# Autodesk Inventor assembly: armAssembaly
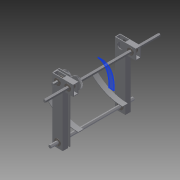
[picture p0: Inventor's stored thumbnail of the model, 180x180]
Saved by Autodesk Inventor 2016 (Build 200138000, 138)
## iProperties
Created: 2016-01-27
Part Number: armAssembaly
Document SubType Name: Assembly
Designer: 278648
Author: 278648
## Documents named in this file (10)
- C:\Users\zachary\Downloads\1510-stronghold-CAD-master\1510-stronghold-CAD-master\pickeruperthingy\armAssembaly.iam
- C:\Users\zachary\Downloads\1510-stronghold-CAD-master\1510-stronghold-CAD-master\pickeruperthingy\arm.ipt
- C:\Users\zachary\Downloads\1510-stronghold-CAD-master\1510-stronghold-CAD-master\pickeruperthingy\217-3875-STEP-20140818.ipt
- C:\Users\zachary\Downloads\1510-stronghold-CAD-master\1510-stronghold-CAD-master\pickeruperthingy\rod.ipt
- C:\Users\zachary\Downloads\1510-stronghold-CAD-master\1510-stronghold-CAD-master\pickeruperthingy\rod2.ipt
- C:\Users\zachary\Downloads\1510-stronghold-CAD-master\1510-stronghold-CAD-master\pickeruperthingy\217-2708.20121204.ipt
- C:\Users\zachary\Downloads\1510-stronghold-CAD-master\1510-stronghold-CAD-master\pickeruperthingy\217-3488-STEP.ipt
- C:\Users\zachary\Downloads\1510-stronghold-CAD-master\1510-stronghold-CAD-master\pickeruperthingy\rod3.ipt
- C:\Users\zachary\Downloads\1510-stronghold-CAD-master\1510-stronghold-CAD-master\pickeruperthingy\Part13.ipt
- C:\Users\zachary\Downloads\1510-stronghold-CAD-master\1510-stronghold-CAD-master\pickeruperthingy\chainguard.ipt
## Components (22 placed, 9 different names)
1. arm:1 — Flush:1, Mate:1, Flush:2, Mate:2, Mate:3, Mate:6, Mate:9, Mate:16, Mate:17, Mate:18, Mate:19, Mate:22, Mate:23, Mate:24, Mate:25, Flush:6, Mate:43, Mate:44, Mate:60, Flush:9, Flush:10, Mate:62
2. arm:2 — Flush:1, Mate:1, Flush:2, Mate:4, Mate:5, Mate:7, Mate:8, Mate:12, Mate:13, Mate:14, Mate:15, Flush:3, Flush:11
3. 217-3875-STEP-20140818:1 — Mate:2, Mate:3, Mate:10, Mate:11
4. 217-3875-STEP-20140818:2 — Mate:4, Mate:5
5. 217-3875-STEP-20140818:3 — Mate:7, Mate:8, Mate:52
6. 217-3875-STEP-20140818:4 — Mate:6, Mate:9, Mate:51
7. rod:1 — Mate:10, Mate:11, Flush:3, Mate:34, Mate:35
8. 217-3875-STEP-20140818:5 — Mate:12, Mate:13
9. 217-3875-STEP-20140818:6 — Mate:14, Mate:15
10. 217-3875-STEP-20140818:7 — Mate:18, Mate:19
11. 217-3875-STEP-20140818:8 — Mate:16, Mate:17, Mate:41, Mate:42
12. 217-3875-STEP-20140818:9 — Mate:22, Mate:23
13. 217-3875-STEP-20140818:12 — Mate:24, Mate:25, Mate:30, Mate:31
14. rod2:2 — Mate:30, Mate:31, Mate:32, Mate:33, Mate:56, Mate:57, Flush:12
15. 217-2708.20121204:1 — Mate:32, Mate:33, Mate:44, Flush:12
16. 217-2708.20121204:2 — Mate:34, Mate:35, Mate:43
17. 217-3488-STEP:1 — Flush:7, Mate:56, Mate:57, Mate:62
18. rod3:1 — Mate:41, Mate:42, Flush:6, Mate:58, Mate:59
19. 217-3488-STEP:2 — Flush:7, Mate:58, Mate:59
20. Part13:1 — Mate:51, Mate:53, Flush:8, Flush:11
21. Part13:2 — Mate:52, Mate:53, Flush:8, Mate:61
22. chainguard:1 — Mate:60, Flush:9, Flush:10, Mate:61
## Relationships (53: Mate 43, Flush 10)
- Flush:1: arm:1 ↔ arm:2
- Mate:1 (279.4 mm): arm:1 ↔ arm:2
- Flush:2: arm:1 ↔ arm:2
- Mate:2: arm:1 ↔ 217-3875-STEP-20140818:1
- Mate:3: arm:1 ↔ 217-3875-STEP-20140818:1
- Mate:4: arm:2 ↔ 217-3875-STEP-20140818:2
- Mate:5: arm:2 ↔ 217-3875-STEP-20140818:2
- Mate:6: arm:1 ↔ 217-3875-STEP-20140818:4
- Mate:7: arm:2 ↔ 217-3875-STEP-20140818:3
- Mate:8: arm:2 ↔ 217-3875-STEP-20140818:3
- Mate:9: arm:1 ↔ 217-3875-STEP-20140818:4
- Mate:10: 217-3875-STEP-20140818:1 ↔ rod:1
- Mate:11: 217-3875-STEP-20140818:1 ↔ rod:1
- Mate:12: arm:2 ↔ 217-3875-STEP-20140818:5
- Mate:13: arm:2 ↔ 217-3875-STEP-20140818:5
- Mate:14: arm:2 ↔ 217-3875-STEP-20140818:6
- Mate:15: arm:2 ↔ 217-3875-STEP-20140818:6
- Mate:16: arm:1 ↔ 217-3875-STEP-20140818:8
- Mate:17: arm:1 ↔ 217-3875-STEP-20140818:8
- Mate:18: arm:1 ↔ 217-3875-STEP-20140818:7
- Mate:19: arm:1 ↔ 217-3875-STEP-20140818:7
- Mate:22: arm:1 ↔ 217-3875-STEP-20140818:9
- Mate:23: arm:1 ↔ 217-3875-STEP-20140818:9
- Mate:24: arm:1 ↔ 217-3875-STEP-20140818:12
- Mate:25: arm:1 ↔ 217-3875-STEP-20140818:12
- Flush:3 (-114.3 mm): arm:2 ↔ rod:1
- Mate:30: 217-3875-STEP-20140818:12 ↔ rod2:2
- Mate:31: 217-3875-STEP-20140818:12 ↔ rod2:2
- Mate:32: rod2:2 ↔ 217-2708.20121204:1
- Mate:33: rod2:2 ↔ 217-2708.20121204:1
- Mate:34: rod:1 ↔ 217-2708.20121204:2
- Mate:35: rod:1 ↔ 217-2708.20121204:2
- Mate:41: 217-3875-STEP-20140818:8 ↔ rod3:1
- Mate:42: 217-3875-STEP-20140818:8 ↔ rod3:1
- Flush:6 (-38.1 mm): arm:1 ↔ rod3:1
- Mate:43 (12.7 mm): arm:1 ↔ 217-2708.20121204:2
- Mate:44 (12.7 mm): arm:1 ↔ 217-2708.20121204:1
- Flush:7: 217-3488-STEP:1 ↔ 217-3488-STEP:2
- Mate:51: 217-3875-STEP-20140818:4 ↔ Part13:1
- Mate:52: 217-3875-STEP-20140818:3 ↔ Part13:2
- Mate:53 (190.5 mm): Part13:1 ↔ Part13:2
- Flush:8: Part13:1 ↔ Part13:2
- Mate:56: rod2:2 ↔ 217-3488-STEP:1
- Mate:57: rod2:2 ↔ 217-3488-STEP:1
- Mate:58: rod3:1 ↔ 217-3488-STEP:2
- Mate:59: rod3:1 ↔ 217-3488-STEP:2
- Mate:60 (8.255 mm): arm:1 ↔ chainguard:1
- Flush:9: arm:1 ↔ chainguard:1
- Flush:10: arm:1 ↔ chainguard:1
- Mate:61 (13.335 mm): Part13:2 ↔ chainguard:1
- Mate:62 (3.175 mm): arm:1 ↔ 217-3488-STEP:1
- Flush:11 (25.4 mm): arm:2 ↔ Part13:1
- Flush:12 (-3.175 mm): rod2:2 ↔ 217-2708.20121204:1
